# Autodesk Inventor assembly: 3-hole gap
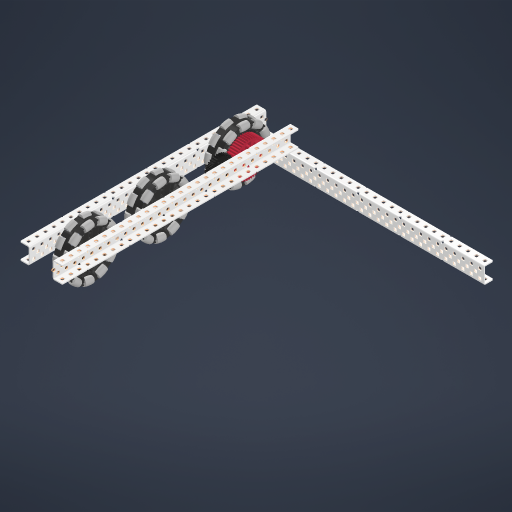
[picture p0: Inventor's stored thumbnail of the model, 512x512]
Saved by Autodesk Inventor 2024.3 (Build 283343000, 343)
## iProperties
Created: 2024-09-26
Part Number: 3-hole gap
Document SubType Name: Assembly
Designer: Juanl
Author: Juanl
## Documents named in this file (7)
- C:\Users\Juanl\Documents\GitHub\ATUM-V5RC-High-Stakes-CAD\Protobot\3-hole gap.iam
- C:\Users\Juanl\Documents\GitHub\ATUM-V5RC-High-Stakes-CAD\VEX-CAD-Inventor\Structure\C Channel\Aluminum 1x2x1\Alu C 1x2x1x28.ipt
- C:\Users\Juanl\Documents\GitHub\ATUM-V5RC-High-Stakes-CAD\VEX-CAD-Inventor\Motion\Wheels\Omni Wheel\3.25 Omni AS, No Insert.iam
- C:\Users\Juanl\Documents\GitHub\ATUM-V5RC-High-Stakes-CAD\VEX-CAD-Inventor\Motion\Wheels\Omni Wheel.iam
- C:\Users\Juanl\Documents\GitHub\ATUM-V5RC-High-Stakes-CAD\VEX-CAD-Inventor\Motion\Gears\HS Gear\HS 48T Gear, No Insert.iam
- C:\Users\Juanl\Documents\GitHub\ATUM-V5RC-High-Stakes-CAD\VEX-CAD-Inventor\Motion\Gears\HS Gear.iam
- C:\Users\Juanl\Documents\GitHub\ATUM-V5RC-High-Stakes-CAD\VEX-CAD-Inventor\Motion\Gears\LS 36T Gear.ipt
## Components (8 placed, 4 different names)
1. Alu C 1x2x1x28:1 — Mate:1, Mate:4, Mate:5
2. Alu C 1x2x1x28:2 — Mate:2, Mate:3, Mate:4, Mate:5, Mate:6, Mate:9
3. Alu C 1x2x1x28:3 — Mate:1, Mate:2, Mate:3
4. 3.25 Omni AS, No Insert:1 [sub-assembly] — Mate:6, Mate:7, Mate:8
5. 3.25 Omni AS, No Insert:2 [sub-assembly]
6. 3.25 Omni AS, No Insert:3 [sub-assembly]
7. HS 48T Gear, No Insert:1 [sub-assembly] — Mate:7, Mate:8
8. LS 36T Gear:1 — Mate:9
## Relationships (9: Mate 9)
- Mate:1: Alu C 1x2x1x28:1 ↔ Alu C 1x2x1x28:3
- Mate:2: Alu C 1x2x1x28:2 ↔ Alu C 1x2x1x28:3
- Mate:3: Alu C 1x2x1x28:2 ↔ Alu C 1x2x1x28:3
- Mate:4: Alu C 1x2x1x28:1 ↔ Alu C 1x2x1x28:2
- Mate:5: Alu C 1x2x1x28:1 ↔ Alu C 1x2x1x28:2
- Mate:6: Alu C 1x2x1x28:2 ↔ 3.25 Omni AS, No Insert:1
- Mate:7: 3.25 Omni AS, No Insert:1 ↔ HS 48T Gear, No Insert:1
- Mate:8: 3.25 Omni AS, No Insert:1 ↔ HS 48T Gear, No Insert:1
- Mate:9: Alu C 1x2x1x28:2 ↔ LS 36T Gear:1
